# Autodesk Inventor assembly: R2 Z-axis Assembly
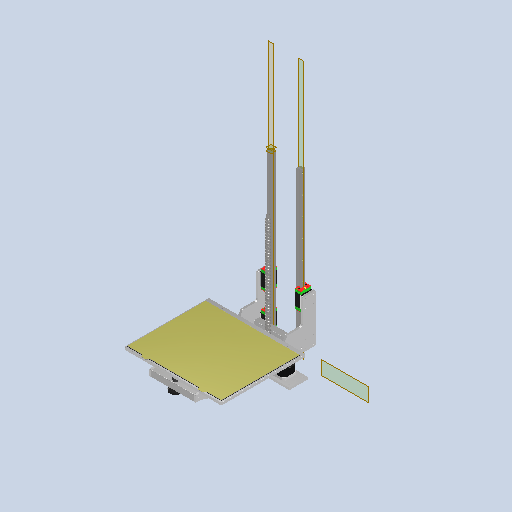
[picture p0: Inventor's stored thumbnail of the model, 512x512]
Saved by Autodesk Inventor 2024 (Build 280153000, 153)
## iProperties
Created: 2024-12-16
Part Number: R2 Z-axis Assembly
Document SubType Name: Assembly
Designer: Ishaan
Author: Ishaan
## Documents named in this file (20)
- E:\Projects\Axiom--IDEX-3D-Printer\CAD\02 - Z-axis\R2 Z-axis Assembly.iam
- E:\Projects\Axiom--IDEX-3D-Printer\CAD\02 - Z-axis\2020 Bed Front Extrusion.ipt
- E:\Projects\Axiom--IDEX-3D-Printer\CAD\02 - Z-axis\Z-Axis Support Plates.ipt
- E:\Projects\Axiom--IDEX-3D-Printer\CAD\02 - Z-axis\2020 Bed Rear Extrusion.ipt
- E:\Projects\Axiom--IDEX-3D-Printer\CAD\02 - Z-axis\4040 Bed Mid Extrusion.ipt
- E:\Projects\Axiom--IDEX-3D-Printer\CAD\00 - COTS Components\HGH15CA Carriage Block\HGH15CA Hiwin Linear block by proma\HGH15CA Hiwin Linear block by proma.ipt
- E:\Projects\Axiom--IDEX-3D-Printer\CAD\00 - COTS Components\Bed Heater\Bed Heater.ipt
- E:\Projects\Axiom--IDEX-3D-Printer\CAD\02 - Z-axis\Print Bed R2.ipt
- E:\Projects\Axiom--IDEX-3D-Printer\CAD\02 - Z-axis\Z-Axis Nut and Bed Plate RevIII.ipt
- E:\Projects\Axiom--IDEX-3D-Printer\CAD\00 - COTS Components\Silicone Bed Spacers\Silicone Bed Spacers.ipt
- E:\Projects\Axiom--IDEX-3D-Printer\CAD\02 - Z-axis\Bed Magnet.ipt
- E:\Projects\Axiom--IDEX-3D-Printer\CAD\02 - Z-axis\PEI Bed Surface.ipt
- E:\Projects\Axiom--IDEX-3D-Printer\CAD\00 - COTS Components\Hardware\M4x12 Spacer.ipt
- E:\Projects\Axiom--IDEX-3D-Printer\CAD\00 - COTS Components\Silicone Bed Spacers\Bed Knob.ipt
- E:\Projects\Axiom--IDEX-3D-Printer\CAD\00 - COTS Components\Hardware\M4x55 Threaded Rod.ipt
- E:\Projects\Axiom--IDEX-3D-Printer\CAD\Rev V Envelope Frame Study.ipt
- E:\Projects\Axiom--IDEX-3D-Printer\CAD\00 - COTS Components\HGR15 Z-Axis Rail\HGR15-R-700mm\R^HGR15-R_0700mm.ipt
- E:\Projects\Axiom--IDEX-3D-Printer\CAD\02 - Z-axis\Z-Axis Nut Plate.ipt
- E:\Projects\Axiom--IDEX-3D-Printer\CAD\00 - COTS Components\1204 Ballscrew Nut\Ballscrew nut 1204 by proma\Ballscrew nut 1204 by proma.ipt
- E:\Projects\Axiom--IDEX-3D-Printer\CAD\02 - Z-axis\Z-axis Drive Assembly.iam
## Components (31 placed, 19 different names)
1. Z-Axis Support Plates:1 — Insert:1, Angle:1, Insert:2, Angle:2, Insert:3, Insert:4, Insert:9, Insert:10, Insert:11, Insert:12, Insert:13, Insert:14, Insert:15, Insert:16, Mate:16
2. 2020 Bed Front Extrusion:1 — Insert:1, Angle:1, Insert:5, Insert:26, Insert:32
3. 2020 Bed Rear Extrusion:1 — Insert:2, Angle:2, Insert:6, Symmetry:1
4. 4040 Bed Mid Extrusion:1 — Insert:3, Insert:4, Insert:7, Insert:8, Mate:1, Flush:3, Mate:2, Symmetry:1, Mate:18, Mate:19
5. Z-Axis Support Plates:2 — Insert:5, Insert:6, Insert:7, Insert:8, Insert:17, Insert:18, Insert:19, Insert:20, Insert:21, Insert:22, Insert:23, Insert:24, Mate:17
6. HGH15CA Hiwin Linear block by proma:1 — Insert:21, Insert:22, Insert:23, Insert:24
7. HGH15CA Hiwin Linear block by proma:2 — Insert:13, Insert:14, Insert:15, Insert:16, Flush:14
8. HGH15CA Hiwin Linear block by proma:3 — Insert:17, Insert:18, Insert:19, Insert:20
9. HGH15CA Hiwin Linear block by proma:4 — Insert:9, Insert:10, Insert:11, Insert:12, Flush:12, Flush:13
10. Bed Heater:1 — Mate:5, Flush:4, Flush:5
11. Print Bed R2:1 — Insert:27, Insert:28, Insert:29, Mate:5, Flush:4, Flush:5, Mate:6, Flush:6, Flush:7, Insert:33, Insert:34, Insert:35
12. Z-Axis Nut and Bed Plate RevIII:1 — Mate:1, Flush:3, Mate:2, Insert:25, Mate:3, Mate:4, Mate:8, Mate:9, Mate:10, Mate:11
13. Silicone Bed Spacers:1 — Mate:3, Mate:4, Insert:28
14. Silicone Bed Spacers:2 — Insert:25, Insert:27
15. Silicone Bed Spacers:3 — Insert:26, Insert:29
16. Bed Magnet:1 — Mate:6, Flush:6, Flush:7, Mate:7, Flush:8, Flush:9
17. PEI Bed Surface:1 — Mate:7, Flush:8, Flush:9
18. M4x12 Spacer:1 — Mate:8, Mate:11, Insert:31
19. M4x12 Spacer:2 — Mate:9, Mate:10, Insert:30
20. Bed Knob:1 — Insert:32
21. Bed Knob:2 — Insert:31
22. Bed Knob:3 — Insert:30
23. M4x55 Threaded Rod:1 — Insert:35
24. M4x55 Threaded Rod:2 — Insert:34
25. M4x55 Threaded Rod:3 — Insert:33
26. Rev V Envelope Frame Study:1 — Mate:12, Mate:13, Mate:14, Mate:15, Mate:16, Mate:17, Angle:3, Mate:21
27. R^HGR15-R_0700mm:1 — Mate:12, Mate:13, Flush:10, Flush:11, Mate:15, Flush:12, Flush:13, Flush:14
28. R^HGR15-R_0700mm:2 — Mate:14, Flush:10, Flush:11
29. Z-Axis Nut Plate:1 — Mate:18, Mate:19, Flush:15, Insert:36, Insert:37
30. Ballscrew nut 1204 by proma:1 — Insert:36, Insert:37, Mate:20
31. Z-axis Drive Assembly:1 [sub-assembly] — Mate:20, Angle:3, Mate:21
## Relationships (75: Insert 37, Mate 21, Flush 13, Angle 3, Symmetry 1)
- Insert:1: Z-Axis Support Plates:1 ↔ 2020 Bed Front Extrusion:1
- Angle:1 (0 deg): Z-Axis Support Plates:1 ↔ 2020 Bed Front Extrusion:1
- Insert:2: Z-Axis Support Plates:1 ↔ 2020 Bed Rear Extrusion:1
- Angle:2 (0 deg): Z-Axis Support Plates:1 ↔ 2020 Bed Rear Extrusion:1
- Insert:3: Z-Axis Support Plates:1 ↔ 4040 Bed Mid Extrusion:1
- Insert:4: Z-Axis Support Plates:1 ↔ 4040 Bed Mid Extrusion:1
- Insert:5: 2020 Bed Front Extrusion:1 ↔ Z-Axis Support Plates:2
- Insert:6: 2020 Bed Rear Extrusion:1 ↔ Z-Axis Support Plates:2
- Insert:7: 4040 Bed Mid Extrusion:1 ↔ Z-Axis Support Plates:2
- Insert:8: 4040 Bed Mid Extrusion:1 ↔ Z-Axis Support Plates:2
- Insert:9: Z-Axis Support Plates:1 ↔ HGH15CA Hiwin Linear block by proma:4
- Insert:10: Z-Axis Support Plates:1 ↔ HGH15CA Hiwin Linear block by proma:4
- Insert:11: Z-Axis Support Plates:1 ↔ HGH15CA Hiwin Linear block by proma:4
- Insert:12: Z-Axis Support Plates:1 ↔ HGH15CA Hiwin Linear block by proma:4
- Insert:13: Z-Axis Support Plates:1 ↔ HGH15CA Hiwin Linear block by proma:2
- Insert:14: Z-Axis Support Plates:1 ↔ HGH15CA Hiwin Linear block by proma:2
- Insert:15: Z-Axis Support Plates:1 ↔ HGH15CA Hiwin Linear block by proma:2
- Insert:16: Z-Axis Support Plates:1 ↔ HGH15CA Hiwin Linear block by proma:2
- Insert:17: Z-Axis Support Plates:2 ↔ HGH15CA Hiwin Linear block by proma:3
- Insert:18: Z-Axis Support Plates:2 ↔ HGH15CA Hiwin Linear block by proma:3
- Insert:19: Z-Axis Support Plates:2 ↔ HGH15CA Hiwin Linear block by proma:3
- Insert:20: Z-Axis Support Plates:2 ↔ HGH15CA Hiwin Linear block by proma:3
- Insert:21: Z-Axis Support Plates:2 ↔ HGH15CA Hiwin Linear block by proma:1
- Insert:22: Z-Axis Support Plates:2 ↔ HGH15CA Hiwin Linear block by proma:1
- Insert:23: Z-Axis Support Plates:2 ↔ HGH15CA Hiwin Linear block by proma:1
- Insert:24: Z-Axis Support Plates:2 ↔ HGH15CA Hiwin Linear block by proma:1
- Mate:1: 4040 Bed Mid Extrusion:1 ↔ Z-Axis Nut and Bed Plate RevIII:1
- Flush:3: 4040 Bed Mid Extrusion:1 ↔ Z-Axis Nut and Bed Plate RevIII:1
- Mate:2: 4040 Bed Mid Extrusion:1 ↔ Z-Axis Nut and Bed Plate RevIII:1
- Insert:25: Z-Axis Nut and Bed Plate RevIII:1 ↔ Silicone Bed Spacers:2
- Insert:26: 2020 Bed Front Extrusion:1 ↔ Silicone Bed Spacers:3
- Mate:3: Z-Axis Nut and Bed Plate RevIII:1 ↔ Silicone Bed Spacers:1
- Mate:4: Z-Axis Nut and Bed Plate RevIII:1 ↔ Silicone Bed Spacers:1
- Insert:27: Print Bed R2:1 ↔ Silicone Bed Spacers:2
- Insert:28: Print Bed R2:1 ↔ Silicone Bed Spacers:1
- Insert:29: Print Bed R2:1 ↔ Silicone Bed Spacers:3
- Mate:5: Bed Heater:1 ↔ Print Bed R2:1
- Flush:4: Bed Heater:1 ↔ Print Bed R2:1
- Flush:5: Bed Heater:1 ↔ Print Bed R2:1
- Mate:6: Print Bed R2:1 ↔ Bed Magnet:1
- Flush:6 (5 mm): Print Bed R2:1 ↔ Bed Magnet:1
- Flush:7 (-5 mm): Print Bed R2:1 ↔ Bed Magnet:1
- Mate:7: Bed Magnet:1 ↔ PEI Bed Surface:1
- Flush:8: Bed Magnet:1 ↔ PEI Bed Surface:1
- Flush:9: Bed Magnet:1 ↔ PEI Bed Surface:1
- Mate:8: Z-Axis Nut and Bed Plate RevIII:1 ↔ M4x12 Spacer:1
- Mate:9: Z-Axis Nut and Bed Plate RevIII:1 ↔ M4x12 Spacer:2
- Mate:10: Z-Axis Nut and Bed Plate RevIII:1 ↔ M4x12 Spacer:2
- Mate:11: Z-Axis Nut and Bed Plate RevIII:1 ↔ M4x12 Spacer:1
- Insert:30: M4x12 Spacer:2 ↔ Bed Knob:3
- Insert:31: M4x12 Spacer:1 ↔ Bed Knob:2
- Insert:32: 2020 Bed Front Extrusion:1 ↔ Bed Knob:1
- Insert:33: Print Bed R2:1 ↔ M4x55 Threaded Rod:3
- Insert:34: Print Bed R2:1 ↔ M4x55 Threaded Rod:2
- Insert:35: Print Bed R2:1 ↔ M4x55 Threaded Rod:1
- Mate:12: Rev V Envelope Frame Study:1 ↔ R^HGR15-R_0700mm:1
- Mate:13 (-10 mm): Rev V Envelope Frame Study:1 ↔ R^HGR15-R_0700mm:1
- Mate:14: Rev V Envelope Frame Study:1 ↔ R^HGR15-R_0700mm:2
- Flush:10: R^HGR15-R_0700mm:1 ↔ R^HGR15-R_0700mm:2
- Flush:11: R^HGR15-R_0700mm:1 ↔ R^HGR15-R_0700mm:2
- Mate:15 (40 mm): Rev V Envelope Frame Study:1 ↔ R^HGR15-R_0700mm:1
- Mate:16 (28 mm): Z-Axis Support Plates:1 ↔ Rev V Envelope Frame Study:1
- Mate:17 (28 mm): Z-Axis Support Plates:2 ↔ Rev V Envelope Frame Study:1
- Flush:12: HGH15CA Hiwin Linear block by proma:4 ↔ R^HGR15-R_0700mm:1
- Flush:13: HGH15CA Hiwin Linear block by proma:4 ↔ R^HGR15-R_0700mm:1
- Flush:14: HGH15CA Hiwin Linear block by proma:2 ↔ R^HGR15-R_0700mm:1
- Symmetry:1: 2020 Bed Rear Extrusion:1 ↔ 4040 Bed Mid Extrusion:1
- Mate:18: 4040 Bed Mid Extrusion:1 ↔ Z-Axis Nut Plate:1
- Mate:19: 4040 Bed Mid Extrusion:1 ↔ Z-Axis Nut Plate:1
- Flush:15: Z-Axis Nut Plate:1
- Insert:36: Z-Axis Nut Plate:1 ↔ Ballscrew nut 1204 by proma:1
- Insert:37: Z-Axis Nut Plate:1 ↔ Ballscrew nut 1204 by proma:1
- Mate:20: Ballscrew nut 1204 by proma:1 ↔ Z-axis Drive Assembly:1
- Angle:3 (0 deg): Rev V Envelope Frame Study:1 ↔ Z-axis Drive Assembly:1
- Mate:21: Rev V Envelope Frame Study:1 ↔ Z-axis Drive Assembly:1
